# Autodesk Inventor assembly: UpperArmActuatorBase
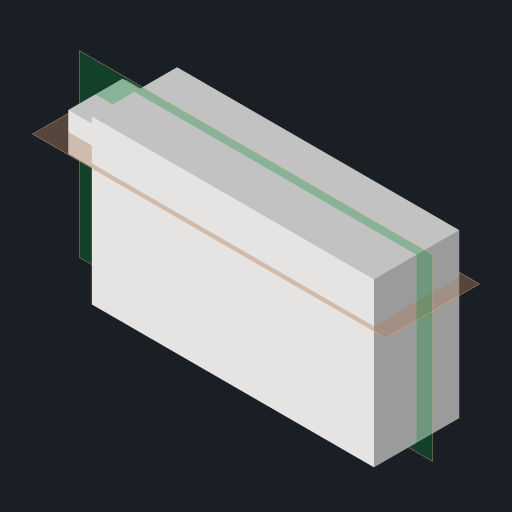
[picture p0: Inventor's stored thumbnail of the model, 512x512]
Saved by Autodesk Inventor 2023 (Build 270158000, 158)
## iProperties
Created: 2023-03-23
Part Number: UpperArmActuatorBase
Document SubType Name: Assembly
Designer: Val
Author: Val
## Documents named in this file (3)
- C:\Users\valer\Desktop\str1ker\cad\external\UpperArmActuator\UpperArmActuatorBase.iam
- C:\Users\valer\Desktop\str1ker\cad\external\UpperArmActuator\UpperArmActuatorBody.ipt
- C:\Users\valer\Desktop\str1ker\cad\external\UpperArmActuator\UpperArmActuatorBaseBoundingBox.ipt
## Components (2 placed, 2 different names)
1. UpperArmActuatorBody:1 — Mate:1, Flush:4, Angle:1, Mate:2, Flush:6
2. UpperArmActuatorBaseBoundingBox:1 — Mate:2, Flush:5, Flush:6
## Relationships (6: Flush 3, Mate 2, Angle 1)
- Mate:1: UpperArmActuatorBody:1
- Flush:4: UpperArmActuatorBody:1
- Angle:1 (0 deg): UpperArmActuatorBody:1
- Mate:2: UpperArmActuatorBody:1 ↔ UpperArmActuatorBaseBoundingBox:1
- Flush:5: UpperArmActuatorBaseBoundingBox:1
- Flush:6: UpperArmActuatorBody:1 ↔ UpperArmActuatorBaseBoundingBox:1
